# Autodesk Inventor assembly: MechSwitch_Assembly
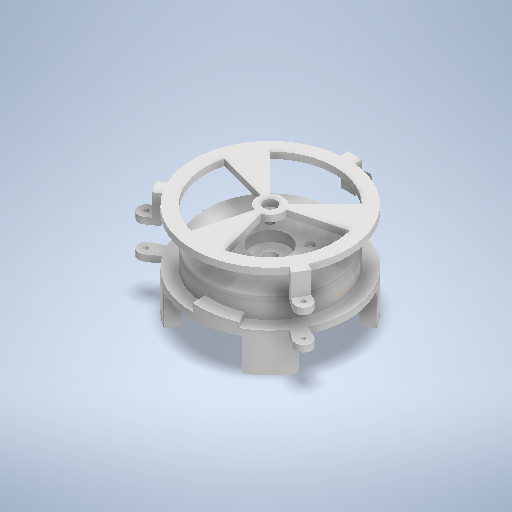
[picture p0: Inventor's stored thumbnail of the model, 512x512]
Saved by Autodesk Inventor 2025.1 (Build 291241000, 241)
## iProperties
Created: 2026-02-23
Part Number: MechSwitch_Assembly
Document SubType Name: Assembly
Designer: ryand
Author: ryand
## Documents named in this file (3)
- C:\Users\ryand\OneDrive\Documents\Inventor\TNG\Rotational_TENG\MechSwitch\MechSwitch_Assembly.iam
- C:\Users\ryand\OneDrive\Documents\Inventor\TNG\Rotational_TENG\MechSwitch\MechSwitch_DielecTop.ipt
- C:\Users\ryand\OneDrive\Documents\Inventor\TNG\Rotational_TENG\MechSwitch\MechSwitch_MotorBaseiptV1.ipt
## Components (2 placed, 2 different names)
1. MechSwitch_DielecTop:1 — Insert:1
2. MechSwitch_MotorBaseiptV1:1 — Insert:1
## Relationships (1: Insert 1)
- Insert:1 (20 mm): MechSwitch_DielecTop:1 ↔ MechSwitch_MotorBaseiptV1:1
